# Autodesk Inventor assembly: Shooter Curve Assembly
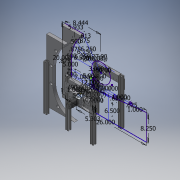
[picture p0: Inventor's stored thumbnail of the model, 180x180]
Saved by Autodesk Inventor 2018 (Build 220112000, 112)
## iProperties
Created: 2020-02-01
Part Number: Shooter Curve Assembly
Document SubType Name: Assembly
Designer: Weeb No1
Author: Weeb No1
## Documents named in this file (8)
- C:\Users\Weeb No1\Documents\GitHub\2020CAD\Gabriel Inventor Files (Shooter, Drivebase)\Shooter Curve Assembly\Main Assembly File\Shooter Curve Assembly.iam
- C:\Users\Weeb No1\Documents\GitHub\2020CAD\Gabriel Inventor Files (Shooter, Drivebase)\Shooter Curve Assembly\Part Files\Shooter Main Curve.ipt
- C:\Users\Weeb No1\Documents\GitHub\2020CAD\Gabriel Inventor Files (Shooter, Drivebase)\Shooter Curve Assembly\Part Files\8020 1010 x 13.ipt
- C:\Users\Weeb No1\Documents\GitHub\2020CAD\Gabriel Inventor Files (Shooter, Drivebase)\Shooter Curve Assembly\Part Files\1x2 5 in Beam Flywheel Mount.ipt
- C:\Users\Weeb No1\Documents\GitHub\2020CAD\Over bumper intake\Parts\VersaPlanetary_v2_Single_Stage_10_1_with_775_Series.iam
- C:\Users\Weeb No1\Documents\GitHub\2020CAD\Gabriel Inventor Files (Shooter, Drivebase)\Shooter Curve Assembly\Part Files\1x2 2 625 in Beam Flywheel Mount.ipt
- C:\Users\Weeb No1\Documents\GitHub\2020CAD\Gabriel Inventor Files (Shooter, Drivebase)\Drivebase Assembly\Part Files\L-Bracket v1.ipt
- C:\Users\Weeb No1\Documents\GitHub\2020CAD\Gabriel Inventor Files (Shooter, Drivebase)\Drivebase Assembly\Part Files\L-Guesset v1.ipt
## Components (23 placed, 7 different names)
1. Shooter Main Curve:1 — Flush:1, Mate:1, Mate:2, Flush:2, Flush:3, Flush:18, Flush:20, Flush:30, Mate:15, Flush:32, Flush:33
2. 8020 1010 x 13:1 — Flush:1, Mate:1, Flush:5, Flush:6, Mate:7, Flush:11, Flush:14, Flush:18, Flush:23, Flush:24, Mate:17, Flush:35
3. 8020 1010 x 13:2 — Flush:4, Mate:3, Flush:7, Mate:9, Flush:15, Flush:19, Flush:22, Flush:25
4. Shooter Main Curve:2 — Mate:2, Flush:2, Flush:3, Flush:4, Mate:3, Flush:19, Flush:21, Mate:14, Flush:31
5. 8020 1010 x 13:3 — Flush:5, Flush:6, Flush:10, Flush:12, Flush:13, Flush:20, Mate:11, Flush:23, Mate:12, Flush:28, Flush:29, Mate:16, Flush:34, Mate:35
6. 8020 1010 x 13:4 — Flush:7, Flush:10, Flush:17, Flush:21, Mate:10, Flush:22, Mate:13, Flush:26, Flush:27
7. 1x2 5 in Beam Flywheel Mount:1 — Mate:9, Flush:15, Flush:17, Mate:10, Flush:25, Mate:40, Mate:41, Mate:42, Mate:43, Mate:44, Mate:45
8. 1x2 5 in Beam Flywheel Mount:2 — Mate:7, Flush:11, Flush:12, Flush:13, Flush:14, Mate:11, Flush:24, Mate:37, Mate:38, Mate:39
9. 8020 1010 x 13:5 — Mate:13, Flush:26, Flush:27
10. 8020 1010 x 13:6 — Mate:12, Flush:28, Flush:29
11. 8020 1010 x 13:7 — Flush:30, Mate:14, Flush:31
12. 8020 1010 x 13:8 — Mate:15, Flush:32, Flush:33
13. VersaPlanetary_v2_Single_Stage_10_1_with_775_Series:1 [sub-assembly] — Mate:18, Mate:19, Mate:20, Mate:21, Mate:24, Mate:25, Mate:27, Mate:28, Mate:31, Mate:32
14. 1x2 2 625 in Beam Flywheel Mount:1 — Mate:17, Flush:35, Flush:36, Mate:19, Mate:22, Mate:23, Mate:33
15. 1x2 2 625 in Beam Flywheel Mount:2 — Mate:16, Flush:34, Flush:36, Mate:18, Mate:26, Mate:29, Mate:36
16. L-Bracket v1:1 — Mate:20, Mate:21, Mate:22, Mate:23, Mate:34
17. L-Bracket v1:2 — Mate:24, Mate:25, Mate:26, Mate:30
18. L-Bracket v1:3 — Mate:27, Mate:28, Mate:29, Mate:30
19. L-Bracket v1:4 — Mate:31, Mate:32, Mate:33, Mate:34
20. L-Guesset v1:1 — Mate:40, Mate:41, Mate:42
21. L-Guesset v1:2 — Mate:43, Mate:44, Mate:45
22. L-Guesset v1:3 — Mate:37, Mate:38, Mate:39
23. L-Guesset v1:4 — Mate:35, Mate:36
## Relationships (74: Mate 41, Flush 33)
- Flush:1 (203.2 mm): Shooter Main Curve:1 ↔ 8020 1010 x 13:1
- Mate:1 (25.4 mm): Shooter Main Curve:1 ↔ 8020 1010 x 13:1
- Mate:2 (101.6 mm): Shooter Main Curve:1 ↔ Shooter Main Curve:2
- Flush:2: Shooter Main Curve:1 ↔ Shooter Main Curve:2
- Flush:3: Shooter Main Curve:1 ↔ Shooter Main Curve:2
- Flush:4 (203.2 mm): 8020 1010 x 13:2 ↔ Shooter Main Curve:2
- Mate:3 (25.4 mm): 8020 1010 x 13:2 ↔ Shooter Main Curve:2
- Flush:5: 8020 1010 x 13:1 ↔ 8020 1010 x 13:3
- Flush:6: 8020 1010 x 13:1 ↔ 8020 1010 x 13:3
- Flush:7: 8020 1010 x 13:2 ↔ 8020 1010 x 13:4
- Flush:10: 8020 1010 x 13:3 ↔ 8020 1010 x 13:4
- Mate:7: 8020 1010 x 13:1 ↔ 1x2 5 in Beam Flywheel Mount:2
- Flush:11: 8020 1010 x 13:1 ↔ 1x2 5 in Beam Flywheel Mount:2
- Flush:12: 8020 1010 x 13:3 ↔ 1x2 5 in Beam Flywheel Mount:2
- Flush:13: 8020 1010 x 13:3 ↔ 1x2 5 in Beam Flywheel Mount:2
- Flush:14: 8020 1010 x 13:1 ↔ 1x2 5 in Beam Flywheel Mount:2
- Mate:9: 8020 1010 x 13:2 ↔ 1x2 5 in Beam Flywheel Mount:1
- Flush:15: 8020 1010 x 13:2 ↔ 1x2 5 in Beam Flywheel Mount:1
- Flush:17: 8020 1010 x 13:4 ↔ 1x2 5 in Beam Flywheel Mount:1
- Flush:18 (-37.846 mm): Shooter Main Curve:1 ↔ 8020 1010 x 13:1
- Flush:19 (-37.846 mm): 8020 1010 x 13:2 ↔ Shooter Main Curve:2
- Flush:20 (-37.846 mm): Shooter Main Curve:1 ↔ 8020 1010 x 13:3
- Flush:21 (-37.846 mm): Shooter Main Curve:2 ↔ 8020 1010 x 13:4
- Mate:10: 8020 1010 x 13:4 ↔ 1x2 5 in Beam Flywheel Mount:1
- Mate:11: 8020 1010 x 13:3 ↔ 1x2 5 in Beam Flywheel Mount:2
- Flush:22: 8020 1010 x 13:2 ↔ 8020 1010 x 13:4
- Flush:23: 8020 1010 x 13:1 ↔ 8020 1010 x 13:3
- Flush:24: 8020 1010 x 13:1 ↔ 1x2 5 in Beam Flywheel Mount:2
- Flush:25: 8020 1010 x 13:2 ↔ 1x2 5 in Beam Flywheel Mount:1
- Mate:12 (127 mm): 8020 1010 x 13:3 ↔ 8020 1010 x 13:6
- Mate:13 (127 mm): 8020 1010 x 13:4 ↔ 8020 1010 x 13:5
- Flush:26: 8020 1010 x 13:4 ↔ 8020 1010 x 13:5
- Flush:27: 8020 1010 x 13:4 ↔ 8020 1010 x 13:5
- Flush:28: 8020 1010 x 13:3 ↔ 8020 1010 x 13:6
- Flush:29: 8020 1010 x 13:3 ↔ 8020 1010 x 13:6
- Flush:30: Shooter Main Curve:1 ↔ 8020 1010 x 13:7
- Mate:14: Shooter Main Curve:2 ↔ 8020 1010 x 13:7
- Flush:31 (-37.846 mm): Shooter Main Curve:2 ↔ 8020 1010 x 13:7
- Mate:15: Shooter Main Curve:1 ↔ 8020 1010 x 13:8
- Flush:32: Shooter Main Curve:1 ↔ 8020 1010 x 13:8
- Flush:33 (-37.846 mm): Shooter Main Curve:1 ↔ 8020 1010 x 13:8
- Mate:16: 8020 1010 x 13:3 ↔ 1x2 2 625 in Beam Flywheel Mount:2
- Flush:34: 8020 1010 x 13:3 ↔ 1x2 2 625 in Beam Flywheel Mount:2
- Mate:17: 8020 1010 x 13:1 ↔ 1x2 2 625 in Beam Flywheel Mount:1
- Flush:35: 8020 1010 x 13:1 ↔ 1x2 2 625 in Beam Flywheel Mount:1
- Flush:36: 1x2 2 625 in Beam Flywheel Mount:1 ↔ 1x2 2 625 in Beam Flywheel Mount:2
- Mate:18: VersaPlanetary_v2_Single_Stage_10_1_with_775_Series:1 ↔ 1x2 2 625 in Beam Flywheel Mount:2
- Mate:19: VersaPlanetary_v2_Single_Stage_10_1_with_775_Series:1 ↔ 1x2 2 625 in Beam Flywheel Mount:1
- Mate:20: VersaPlanetary_v2_Single_Stage_10_1_with_775_Series:1 ↔ L-Bracket v1:1
- Mate:21: VersaPlanetary_v2_Single_Stage_10_1_with_775_Series:1 ↔ L-Bracket v1:1
- Mate:22: 1x2 2 625 in Beam Flywheel Mount:1 ↔ L-Bracket v1:1
- Mate:23: 1x2 2 625 in Beam Flywheel Mount:1 ↔ L-Bracket v1:1
- Mate:24: VersaPlanetary_v2_Single_Stage_10_1_with_775_Series:1 ↔ L-Bracket v1:2
- Mate:25: VersaPlanetary_v2_Single_Stage_10_1_with_775_Series:1 ↔ L-Bracket v1:2
- Mate:26: 1x2 2 625 in Beam Flywheel Mount:2 ↔ L-Bracket v1:2
- Mate:27: VersaPlanetary_v2_Single_Stage_10_1_with_775_Series:1 ↔ L-Bracket v1:3
- Mate:28: VersaPlanetary_v2_Single_Stage_10_1_with_775_Series:1 ↔ L-Bracket v1:3
- Mate:29: 1x2 2 625 in Beam Flywheel Mount:2 ↔ L-Bracket v1:3
- Mate:30: L-Bracket v1:2 ↔ L-Bracket v1:3
- Mate:31: VersaPlanetary_v2_Single_Stage_10_1_with_775_Series:1 ↔ L-Bracket v1:4
- Mate:32: VersaPlanetary_v2_Single_Stage_10_1_with_775_Series:1 ↔ L-Bracket v1:4
- Mate:33: 1x2 2 625 in Beam Flywheel Mount:1 ↔ L-Bracket v1:4
- Mate:34: L-Bracket v1:1 ↔ L-Bracket v1:4
- Mate:35: 8020 1010 x 13:3 ↔ L-Guesset v1:4
- Mate:36: 1x2 2 625 in Beam Flywheel Mount:2 ↔ L-Guesset v1:4
- Mate:37: 1x2 5 in Beam Flywheel Mount:2 ↔ L-Guesset v1:3
- Mate:38: 1x2 5 in Beam Flywheel Mount:2 ↔ L-Guesset v1:3
- Mate:39: 1x2 5 in Beam Flywheel Mount:2 ↔ L-Guesset v1:3
- Mate:40: 1x2 5 in Beam Flywheel Mount:1 ↔ L-Guesset v1:1
- Mate:41: 1x2 5 in Beam Flywheel Mount:1 ↔ L-Guesset v1:1
- Mate:42: 1x2 5 in Beam Flywheel Mount:1 ↔ L-Guesset v1:1
- Mate:43: 1x2 5 in Beam Flywheel Mount:1 ↔ L-Guesset v1:2
- Mate:44: 1x2 5 in Beam Flywheel Mount:1 ↔ L-Guesset v1:2
- Mate:45: 1x2 5 in Beam Flywheel Mount:1 ↔ L-Guesset v1:2
